# Autodesk Inventor assembly: printer
(part 2 of 2)
- Mate:177: CSN 02 1702 B B 4,3:115 ↔ ISO 4762 M4 x 20:64
- Mate:178: z_rod_stopper_bottom:2 ↔ CSN 02 1702 B B 4,3:119
- Mate:179: CSN 02 1702 B B 4,3:119 ↔ ISO 4762 M4 x 20:63
- Mate:180: z_motor_mount:2 ↔ CSN 02 1702 B B 4,3:128
- Mate:181: CSN 02 1702 B B 4,3:128 ↔ ISO 4762 M4 x 20:60
- Mate:182: z_motor_mount:2 ↔ CSN 02 1702 B B 4,3:118
- Mate:183: CSN 02 1702 B B 4,3:118 ↔ ISO 4762 M4 x 20:58
- Mate:184: brace_right:1 ↔ CSN 02 1702 B B 4,3:126
- Mate:185: CSN 02 1702 B B 4,3:126 ↔ ISO 4762 M4 x 20:62
- Mate:186: z_rod_stopper_bottom:2 ↔ CSN 02 1702 B B 4,3:127
- Mate:187: CSN 02 1702 B B 4,3:127 ↔ ISO 4762 M4 x 20:61
- Mate:188: CSN 02 1702 B B 4,3:119 ↔ DIN EN ISO 7040 M4:51
- Mate:189: ISO 4762 M4 x 20:63 ↔ DIN EN ISO 7040 M4:51
- Mate:190: CSN 02 1702 B B 4,3:115 ↔ DIN EN ISO 7040 M4:54
- Mate:191: ISO 4762 M4 x 20:64 ↔ DIN EN ISO 7040 M4:54
- Mate:192: CSN 02 1702 B B 4,3:125 ↔ DIN EN ISO 7040 M4:52
- Mate:193: ISO 4762 M4 x 20:59 ↔ DIN EN ISO 7040 M4:52
- Mate:194: CSN 02 1702 B B 4,3:128 ↔ DIN EN ISO 7040 M4:53
- Mate:195: ISO 4762 M4 x 20:60 ↔ DIN EN ISO 7040 M4:53
- Mate:196: CSN 02 1702 B B 4,3:118 ↔ DIN EN ISO 7040 M4:55
- Mate:197: ISO 4762 M4 x 20:58 ↔ DIN EN ISO 7040 M4:55
- Mate:198: CSN 02 1702 B B 4,3:126 ↔ DIN EN ISO 7040 M4:50
- Mate:199: ISO 4762 M4 x 20:62 ↔ DIN EN ISO 7040 M4:50
- Mate:200: CSN 02 1702 B B 4,3:127 ↔ DIN EN ISO 7040 M4:49
- Mate:201: ISO 4762 M4 x 20:61 ↔ DIN EN ISO 7040 M4:49
- Mate:202: brace_right:1 ↔ wiring_brace:1
- Mate:203: frame:1 ↔ wiring_brace:1
- Mate:204: brace_right:1 ↔ wiring_brace:1
- Mate:205: brace_left:1 ↔ wiring_brace:2
- Mate:206: frame:1 ↔ wiring_brace:2
- Mate:207: brace_left:1 ↔ wiring_brace:2
- Mate:208: frame:1 ↔ CSN 02 1702 B B 4,3:132
- Mate:209: frame:1 ↔ CSN 02 1702 B B 4,3:132
- Mate:210: wiring_brace:1 ↔ CSN 02 1702 B B 4,3:131
- Mate:211: brace_right:1 ↔ CSN 02 1702 B B 4,3:129
- Mate:212: brace_right:1 ↔ CSN 02 1702 B B 4,3:129
- Mate:213: wiring_brace:1 ↔ CSN 02 1702 B B 4,3:130
- Insert:30: CSN 02 1702 B B 4,3:132 ↔ ISO 4762 M4 x 20:65
- Insert:31: CSN 02 1702 B B 4,3:129 ↔ ISO 4762 M4 x 20:66
- Mate:214: CSN 02 1702 B B 4,3:131 ↔ ISO 4762 M4 x 20:65
- Mate:215: CSN 02 1702 B B 4,3:130 ↔ ISO 4762 M4 x 20:66
- Mate:216: CSN 02 1702 B B 4,3:131 ↔ DIN EN ISO 7040 M4:57
- Mate:217: ISO 4762 M4 x 20:65 ↔ DIN EN ISO 7040 M4:57
- Mate:218: CSN 02 1702 B B 4,3:130 ↔ DIN EN ISO 7040 M4:56
- Mate:219: ISO 4762 M4 x 20:66 ↔ DIN EN ISO 7040 M4:56
- Mate:220: z_motor_mount:2 ↔ CSN 02 1702 B B 3,2:3
- Mate:221: z_motor_mount:2 ↔ CSN 02 1702 B B 3,2:2
- Mate:222: z_motor_mount:2 ↔ CSN 02 1702 B B 3,2:1
- Mate:223: z_motor_mount:2 ↔ CSN 02 1702 B B 3,2:4
- Mate:224: z_motor_mount:2 ↔ CSN 02 1702 B B 3,2:2
- Mate:225: z_motor_mount:2 ↔ CSN 02 1702 B B 3,2:4
- Mate:226: z_motor_mount:2 ↔ CSN 02 1702 B B 3,2:3
- Mate:227: z_motor_mount:2 ↔ CSN 02 1702 B B 3,2:1
- Insert:32: CSN 02 1702 B B 3,2:4 ↔ ISO 4762 M3 x 16:2
- Insert:33: CSN 02 1702 B B 3,2:2 ↔ ISO 4762 M3 x 16:1
- Insert:34: CSN 02 1702 B B 3,2:3 ↔ ISO 4762 M3 x 16:3
- Insert:35: CSN 02 1702 B B 3,2:1 ↔ ISO 4762 M3 x 16:4
- Mate:228: CSN 02 1702 B B 4,3:136 ↔ ISO 4762 M4 x 20:67
- Insert:36: CSN 02 1702 B B 4,3:142 ↔ ISO 4762 M4 x 20:67
- Mate:229: CSN 02 1702 B B 4,3:143 ↔ ISO 4762 M4 x 20:68
- Insert:37: CSN 02 1702 B B 4,3:135 ↔ ISO 4762 M4 x 20:68
- Mate:230: CSN 02 1702 B B 4,3:146 ↔ ISO 4762 M4 x 20:69
- Insert:38: CSN 02 1702 B B 4,3:141 ↔ ISO 4762 M4 x 20:69
- Mate:231: CSN 02 1702 B B 4,3:145 ↔ ISO 4762 M4 x 20:70
- Insert:39: CSN 02 1702 B B 4,3:140 ↔ ISO 4762 M4 x 20:70
- Mate:232: CSN 02 1702 B B 4,3:144 ↔ ISO 4762 M4 x 20:71
- Insert:40: CSN 02 1702 B B 4,3:134 ↔ ISO 4762 M4 x 20:71
- Mate:233: CSN 02 1702 B B 4,3:137 ↔ ISO 4762 M4 x 20:72
- Insert:41: CSN 02 1702 B B 4,3:139 ↔ ISO 4762 M4 x 20:72
- Mate:234: CSN 02 1702 B B 4,3:133 ↔ ISO 4762 M4 x 20:73
- Insert:42: CSN 02 1702 B B 4,3:138 ↔ ISO 4762 M4 x 20:73
- Mate:235: ISO 4762 M4 x 20:70 ↔ DIN EN ISO 7040 M4:58
- Mate:236: CSN 02 1702 B B 4,3:145 ↔ DIN EN ISO 7040 M4:58
- Mate:237: ISO 4762 M4 x 20:71 ↔ DIN EN ISO 7040 M4:59
- Mate:238: CSN 02 1702 B B 4,3:144 ↔ DIN EN ISO 7040 M4:59
- Mate:239: ISO 4762 M4 x 20:72 ↔ DIN EN ISO 7040 M4:60
- Mate:240: CSN 02 1702 B B 4,3:137 ↔ DIN EN ISO 7040 M4:60
- Mate:241: ISO 4762 M4 x 20:68 ↔ DIN EN ISO 7040 M4:61
- Mate:242: CSN 02 1702 B B 4,3:143 ↔ DIN EN ISO 7040 M4:61
- Mate:243: ISO 4762 M4 x 20:69 ↔ DIN EN ISO 7040 M4:62
- Mate:244: CSN 02 1702 B B 4,3:146 ↔ DIN EN ISO 7040 M4:62
- Mate:245: ISO 4762 M4 x 20:73 ↔ DIN EN ISO 7040 M4:63
- Mate:246: CSN 02 1702 B B 4,3:133 ↔ DIN EN ISO 7040 M4:63
- Mate:247: ISO 4762 M4 x 20:67 ↔ DIN EN ISO 7040 M4:64
- Mate:248: CSN 02 1702 B B 4,3:136 ↔ DIN EN ISO 7040 M4:64
- Mate:249: CSN 02 1702 B B 4,3:149 ↔ ISO 4762 M4 x 20:74
- Insert:43: CSN 02 1702 B B 4,3:150 ↔ ISO 4762 M4 x 20:74
- Mate:250: CSN 02 1702 B B 4,3:148 ↔ ISO 4762 M4 x 20:75
- Insert:44: CSN 02 1702 B B 4,3:147 ↔ ISO 4762 M4 x 20:75
- Mate:251: ISO 4762 M4 x 20:75 ↔ DIN EN ISO 7040 M4:65
- Mate:252: CSN 02 1702 B B 4,3:148 ↔ DIN EN ISO 7040 M4:65
- Mate:253: ISO 4762 M4 x 20:74 ↔ DIN EN ISO 7040 M4:66
- Mate:254: CSN 02 1702 B B 4,3:149 ↔ DIN EN ISO 7040 M4:66
- Insert:45: CSN 02 1702 B B 3,2:6 ↔ ISO 4762 M3 x 16:5
- Insert:46: CSN 02 1702 B B 3,2:8 ↔ ISO 4762 M3 x 16:6
- Insert:47: CSN 02 1702 B B 3,2:7 ↔ ISO 4762 M3 x 16:7
- Insert:48: CSN 02 1702 B B 3,2:5 ↔ ISO 4762 M3 x 16:8
- Mate:255: back:1 ↔ PC Fan:1
- Mate:256: back:1 ↔ PC Fan:1
- Mate:257: back:1 ↔ PC Fan:1
- Mate:258 (3 mm): back:1 ↔ User Library-Fan Guard:1
- Mate:259: y_carriage_belt_iddler:2 ↔ y_carriage_belt_iddler_holder:1
- Mate:260: y_carriage_belt_iddler:2 ↔ y_carriage_belt_iddler_holder:1
- Mate:261: y_carriage_belt_iddler:2 ↔ y_carriage_belt_iddler_holder:1
- Mate:262: y_carriage_belt_iddler:1 ↔ y_carriage_belt_iddler_holder:1
- Mate:263: y_carriage_belt_iddler:1 ↔ y_carriage_belt_iddler_holder:1
- Mate:264: y_carriage_belt_iddler:1 ↔ y_carriage_belt_iddler_holder:1
- Mate:265: 608RS:1 ↔ belt_guide:1
- Mate:266: 608RS:1 ↔ belt_guide:1
- Mate:267: belt_guide:1 ↔ belt_guide:2
- Mate:268: belt_guide:1 ↔ belt_guide:2
- Mate:269: 608RS:1 ↔ belt_guide:2
- Mate:270: CSN 02 1702 B B 8,4:5 ↔ CSN 02 1702 B B 8,4:6
- Mate:271: CSN 02 1702 B B 8,4:5 ↔ CSN 02 1702 B B 8,4:6
- Mate:272: CSN 02 1702 B B 8,4:3 ↔ CSN 02 1702 B B 8,4:4
- Mate:273: CSN 02 1702 B B 8,4:3 ↔ CSN 02 1702 B B 8,4:4
- Mate:274: 608RS:1 ↔ CSN 02 1702 B B 8,4:4
- Mate:275: 608RS:1 ↔ CSN 02 1702 B B 8,4:4
- Mate:276: 608RS:1 ↔ CSN 02 1702 B B 8,4:5
- Mate:277: 608RS:1 ↔ CSN 02 1702 B B 8,4:5
- Mate:278: y_carriage_belt_iddler:1 ↔ CSN 02 1702 B B 8,4:6
- Mate:279: y_carriage_belt_iddler:2 ↔ 608RS:1
- Mate:280: y_carriage_belt_iddler:2 ↔ CSN 02 1702 B B 8,4:1
- Mate:281: y_carriage_belt_iddler:2 ↔ CSN 02 1702 B B 8,4:1
- Mate:282: y_carriage_belt_iddler:1 ↔ CSN 02 1702 B B 8,4:2
- Mate:283: y_carriage_belt_iddler:1 ↔ CSN 02 1702 B B 8,4:2
- Insert:49: CSN 02 1702 B B 8,4:2 ↔ ISO 4762 M8 x 40:1
- Mate:284: CSN 02 1702 B B 8,4:1 ↔ DIN EN ISO 7040 M8:1
- Mate:285: ISO 4762 M8 x 40:1 ↔ DIN EN ISO 7040 M8:1
- Mate:286: back:1 ↔ y_carriage_belt_iddler:2
- Mate:287: back:1 ↔ y_carriage_belt_iddler:2
- Mate:288: back:1 ↔ y_carriage_belt_iddler:1
- Mate:289: back:1 ↔ CSN 02 1702 B B 4,3:152
- Mate:290: back:1 ↔ CSN 02 1702 B B 4,3:153
- Mate:291: back:1 ↔ CSN 02 1702 B B 4,3:153
- Mate:292: back:1 ↔ CSN 02 1702 B B 4,3:152
- Insert:50: CSN 02 1702 B B 4,3:152 ↔ ISO 4762 M4 x 30:1
- Insert:51: CSN 02 1702 B B 4,3:153 ↔ ISO 4762 M4 x 30:2
- Mate:293: y_carriage_belt_iddler_holder:1 ↔ CSN 02 1702 B B 4,3:154
- Mate:294: y_carriage_belt_iddler_holder:1 ↔ CSN 02 1702 B B 4,3:151
- Mate:295: CSN 02 1702 B B 4,3:151 ↔ ISO 4762 M4 x 30:2
- Mate:296: CSN 02 1702 B B 4,3:154 ↔ ISO 4762 M4 x 30:1
- Mate:297: CSN 02 1702 B B 4,3:151 ↔ DIN EN ISO 7040 M4:68
- Mate:298: ISO 4762 M4 x 30:2 ↔ DIN EN ISO 7040 M4:68
- Mate:299: CSN 02 1702 B B 4,3:154 ↔ DIN EN ISO 7040 M4:67
- Mate:300: ISO 4762 M4 x 30:1 ↔ DIN EN ISO 7040 M4:67
- Mate:301: y_motor_mount:1 ↔ y_motor_mount_brace:1
- Mate:302: y_motor_mount:1 ↔ y_motor_mount_brace:1
- Mate:303: y_motor_mount:1 ↔ y_motor_mount_brace:1
- Mate:304: front:1 ↔ y_motor_mount:1
- Mate:305: front:1 ↔ y_motor_mount_brace:1
- Mate:306: front:1 ↔ y_motor_mount:1
- Mate:307: front:1 ↔ CSN 02 1702 B B 4,3:159
- Mate:308: front:1 ↔ CSN 02 1702 B B 4,3:160
- Mate:309: front:1 ↔ CSN 02 1702 B B 4,3:160
- Mate:310: front:1 ↔ CSN 02 1702 B B 4,3:159
- Mate:311: y_motor_mount:1 ↔ CSN 02 1702 B B 4,3:157
- Mate:312: y_motor_mount:1 ↔ CSN 02 1702 B B 4,3:157
- Insert:52: CSN 02 1702 B B 4,3:160 ↔ ISO 4762 M4 x 20:78
- Insert:53: CSN 02 1702 B B 4,3:159 ↔ ISO 4762 M4 x 20:77
- Insert:54: CSN 02 1702 B B 4,3:157 ↔ ISO 4762 M4 x 20:76
- Mate:313: y_motor_mount_brace:1 ↔ CSN 02 1702 B B 4,3:158
- Mate:314: CSN 02 1702 B B 4,3:158 ↔ ISO 4762 M4 x 20:78
- Mate:315: y_motor_mount_brace:1 ↔ CSN 02 1702 B B 4,3:155
- Mate:316: CSN 02 1702 B B 4,3:155 ↔ ISO 4762 M4 x 20:76
- Mate:317: y_motor_mount:1 ↔ CSN 02 1702 B B 4,3:156
- Mate:318: CSN 02 1702 B B 4,3:156 ↔ ISO 4762 M4 x 20:77
- Mate:319: CSN 02 1702 B B 4,3:156 ↔ DIN EN ISO 7040 M4:70
- Mate:320: ISO 4762 M4 x 20:77 ↔ DIN EN ISO 7040 M4:70
- Mate:321: CSN 02 1702 B B 4,3:158 ↔ DIN EN ISO 7040 M4:69
- Mate:322: ISO 4762 M4 x 20:78 ↔ DIN EN ISO 7040 M4:69
- Mate:323: CSN 02 1702 B B 4,3:155 ↔ DIN EN ISO 7040 M4:71
- Mate:324: ISO 4762 M4 x 20:76 ↔ DIN EN ISO 7040 M4:71
- Mate:325: motor_spacer:1 ↔ NEMA 17 with T5 Pulley:1
- Mate:326: motor_spacer:1 ↔ NEMA 17 with T5 Pulley:1
- Mate:327: motor_spacer:1 ↔ NEMA 17 with T5 Pulley:1
- Mate:328: y_motor_mount:1 ↔ motor_spacer:1
- Tangent:1: y_motor_mount:1 ↔ motor_spacer:1
- Tangent:2: y_motor_mount:1 ↔ motor_spacer:1
- Mate:329: y_motor_mount:1 ↔ CSN 02 1702 B B 3,2:12
- Mate:330: y_motor_mount:1 ↔ CSN 02 1702 B B 3,2:11
- Mate:331: y_motor_mount:1 ↔ CSN 02 1702 B B 3,2:9
- Mate:332: y_motor_mount:1 ↔ CSN 02 1702 B B 3,2:10
- Insert:55: CSN 02 1702 B B 3,2:12 ↔ ISO 4762 M3 x 16:12
- Insert:56: CSN 02 1702 B B 3,2:11 ↔ ISO 4762 M3 x 16:11
- Insert:57: CSN 02 1702 B B 3,2:9 ↔ ISO 4762 M3 x 16:10
- Insert:58: CSN 02 1702 B B 3,2:10 ↔ ISO 4762 M3 x 16:9
- Mate:333: motor_spacer:1 ↔ ISO 4762 M3 x 16:12
- Mate:334: motor_spacer:1 ↔ ISO 4762 M3 x 16:11
- Mate:335: motor_spacer:1 ↔ ISO 4762 M3 x 16:9
- Mate:336: motor_spacer:1 ↔ ISO 4762 M3 x 16:10
- Mate:337: y_axis_rod:2 ↔ y_carryage:1
- Mate:338: y_axis_rod:1 ↔ y_carryage:1
- Mate:339: z_axis_rod:2 ↔ x_axis:1
- Mate:340: z_axis_rod:1 ↔ x_axis:1
- Mate:341: brace_right:1 ↔ CSN 02 1702 B B 4,3:161
- Mate:342: brace_right:1 ↔ CSN 02 1702 B B 4,3:161
- Insert:59: CSN 02 1702 B B 4,3:161 ↔ ISO 4762 M4 x 20:79
- Mate:343: frame_brace_top:1 ↔ CSN 02 1702 B B 4,3:162
- Mate:344: CSN 02 1702 B B 4,3:162 ↔ ISO 4762 M4 x 20:79
- Mate:345: CSN 02 1702 B B 4,3:162 ↔ DIN EN ISO 7040 M4:72
- Mate:346: ISO 4762 M4 x 20:79 ↔ DIN EN ISO 7040 M4:72
- Mate:347: CSN 02 1702 B B 4,3:164 ↔ ISO 4762 M4 x 20:80
- Insert:60: CSN 02 1702 B B 4,3:163 ↔ ISO 4762 M4 x 20:80
- Mate:348: ISO 4762 M4 x 20:80 ↔ DIN EN ISO 7040 M4:73
- Mate:349: CSN 02 1702 B B 4,3:164 ↔ DIN EN ISO 7040 M4:73
- Mate:350: z_axis_top_cap:2 ↔ CSN 02 1702 B B 4,3:172
- Mate:351: z_axis_top_cap:2 ↔ CSN 02 1702 B B 4,3:174
- Mate:352: z_axis_top_cap:2 ↔ CSN 02 1702 B B 4,3:174
- Mate:353: z_axis_top_cap:2 ↔ CSN 02 1702 B B 4,3:172
- Mate:354: z_axis_top:2 ↔ CSN 02 1702 B B 4,3:173
- Mate:355: z_axis_top:2 ↔ CSN 02 1702 B B 4,3:171
- Mate:356: z_axis_top:2 ↔ CSN 02 1702 B B 4,3:170
- Mate:357: z_axis_top:2 ↔ CSN 02 1702 B B 4,3:170
- Mate:358: z_axis_top:2 ↔ CSN 02 1702 B B 4,3:173
- Mate:359: z_axis_top:2 ↔ CSN 02 1702 B B 4,3:171
- Insert:61: CSN 02 1702 B B 4,3:170 ↔ ISO 4762 M4 x 20:81
- Insert:62: CSN 02 1702 B B 4,3:171 ↔ ISO 4762 M4 x 20:82
- Insert:63: CSN 02 1702 B B 4,3:173 ↔ ISO 4762 M4 x 20:83
- Insert:64: CSN 02 1702 B B 4,3:174 ↔ ISO 4762 M4 x 20:84
- Insert:65: CSN 02 1702 B B 4,3:172 ↔ ISO 4762 M4 x 20:85
- Mate:360: brace_right:1 ↔ CSN 02 1702 B B 4,3:169
- Mate:361: CSN 02 1702 B B 4,3:169 ↔ ISO 4762 M4 x 20:81
- Mate:362: frame:1 ↔ CSN 02 1702 B B 4,3:165
- Mate:363: CSN 02 1702 B B 4,3:165 ↔ ISO 4762 M4 x 20:83
- Mate:364: frame:1 ↔ CSN 02 1702 B B 4,3:166
- Mate:365: CSN 02 1702 B B 4,3:166 ↔ ISO 4762 M4 x 20:82
- Mate:366: z_axis_top:2 ↔ CSN 02 1702 B B 4,3:167
- Mate:367: CSN 02 1702 B B 4,3:167 ↔ ISO 4762 M4 x 20:84
- Mate:368: z_axis_top:2 ↔ CSN 02 1702 B B 4,3:168
- Mate:369: CSN 02 1702 B B 4,3:169 ↔ DIN EN ISO 7040 M4:78
- Mate:370: ISO 4762 M4 x 20:81 ↔ DIN EN ISO 7040 M4:78
- Mate:371: CSN 02 1702 B B 4,3:166 ↔ DIN EN ISO 7040 M4:77
- Mate:372: ISO 4762 M4 x 20:82 ↔ DIN EN ISO 7040 M4:77
- Mate:373: CSN 02 1702 B B 4,3:165 ↔ DIN EN ISO 7040 M4:76
- Mate:374: ISO 4762 M4 x 20:83 ↔ DIN EN ISO 7040 M4:76
- Mate:375: CSN 02 1702 B B 4,3:167 ↔ DIN EN ISO 7040 M4:75
- Mate:376: ISO 4762 M4 x 20:84 ↔ DIN EN ISO 7040 M4:75
- Mate:377: CSN 02 1702 B B 4,3:168 ↔ DIN EN ISO 7040 M4:74
- Mate:378: CSN 02 1702 B B 4,3:168 ↔ ISO 4762 M4 x 20:85
- Mate:379: ISO 4762 M4 x 20:85 ↔ DIN EN ISO 7040 M4:74
- Mate:380: CSN 02 1702 B B 4,3:179 ↔ ISO 4762 M4 x 20:86
- Insert:66: CSN 02 1702 B B 4,3:180 ↔ ISO 4762 M4 x 20:86
- Mate:381: CSN 02 1702 B B 4,3:176 ↔ ISO 4762 M4 x 20:87
- Insert:67: CSN 02 1702 B B 4,3:181 ↔ ISO 4762 M4 x 20:87
- Mate:382: CSN 02 1702 B B 4,3:175 ↔ ISO 4762 M4 x 20:88
- Insert:68: CSN 02 1702 B B 4,3:183 ↔ ISO 4762 M4 x 20:88
- Mate:383: CSN 02 1702 B B 4,3:177 ↔ ISO 4762 M4 x 20:89
- Insert:69: CSN 02 1702 B B 4,3:184 ↔ ISO 4762 M4 x 20:89
- Mate:384: CSN 02 1702 B B 4,3:178 ↔ ISO 4762 M4 x 20:90
- Insert:70: CSN 02 1702 B B 4,3:182 ↔ ISO 4762 M4 x 20:90
- Mate:385: ISO 4762 M4 x 20:90 ↔ DIN EN ISO 7040 M4:79
- Mate:386: CSN 02 1702 B B 4,3:178 ↔ DIN EN ISO 7040 M4:79
- Mate:387: ISO 4762 M4 x 20:89 ↔ DIN EN ISO 7040 M4:80
- Mate:388: CSN 02 1702 B B 4,3:177 ↔ DIN EN ISO 7040 M4:80
- Mate:389: ISO 4762 M4 x 20:88 ↔ DIN EN ISO 7040 M4:81
- Mate:390: CSN 02 1702 B B 4,3:175 ↔ DIN EN ISO 7040 M4:81
- Mate:391: ISO 4762 M4 x 20:87 ↔ DIN EN ISO 7040 M4:82
- Mate:392: CSN 02 1702 B B 4,3:176 ↔ DIN EN ISO 7040 M4:82
- Mate:393: ISO 4762 M4 x 20:86 ↔ DIN EN ISO 7040 M4:83
- Mate:394: CSN 02 1702 B B 4,3:179 ↔ DIN EN ISO 7040 M4:83
- Mate:484: bottom:1 ↔ CSN 02 1702 B B 4,3:213
- Mate:485: bottom:1 ↔ CSN 02 1702 B B 4,3:213
- Insert:85: CSN 02 1702 B B 4,3:213 ↔ ISO 4762 M4 x 20:105
- Mate:486: y_motor_mount:1 ↔ CSN 02 1702 B B 4,3:214
- Mate:487: CSN 02 1702 B B 4,3:214 ↔ ISO 4762 M4 x 20:105
- Mate:488: CSN 02 1702 B B 4,3:214 ↔ DIN EN ISO 7040 M4:98
- Mate:489: ISO 4762 M4 x 20:105 ↔ DIN EN ISO 7040 M4:98
- Mate:500: brace_right:1 ↔ IEC inlet:1
- Mate:501: brace_right:1 ↔ IEC inlet:1
- Mate:502: brace_right:1 ↔ IEC inlet:1
- Mate:503: x_axis:1 ↔ z_axis_cable_mount_b:1
- Mate:504: x_axis:1 ↔ z_axis_cable_mount_b:1
- Mate:505: x_axis:1 ↔ z_axis_cable_mount_b:1
- [Insert]: cable_chain_22:28 ↔ cable_chain_22:29
- [Angle] (-36 deg): cable_chain_22:28 ↔ cable_chain_22:29
- [Insert]: cable_chain_22:29 ↔ cable_chain_22:30
- [Angle] (-36 deg): cable_chain_22:29 ↔ cable_chain_22:30
- [Insert]: cable_chain_22:31 ↔ cable_chain_22:32
- [Angle] (-36 deg): cable_chain_22:31 ↔ cable_chain_22:32
- [Insert]: cable_chain_22:32 ↔ cable_chain_22:33
- [Angle] (-36 deg): cable_chain_22:32 ↔ cable_chain_22:33
- [Insert]: cable_chain_22:34 ↔ cable_chain_22:35
- [Angle] (-36 deg): cable_chain_22:34 ↔ cable_chain_22:35
- [Insert]: cable_chain_22:35 ↔ cable_chain_22:36
- [Angle] (-36 deg): cable_chain_22:35 ↔ cable_chain_22:36
- [Insert]: cable_chain_22:33 ↔ cable_chain_22:34
- [Angle] (-36 deg): cable_chain_22:33 ↔ cable_chain_22:34
- [Insert]: cable_chain_22:30 ↔ cable_chain_22:31
- [Angle] (-36 deg): cable_chain_22:30 ↔ cable_chain_22:31
- [Insert]: cable_chain_22:37 ↔ cable_chain_22:38
- [Angle] (-36 deg): cable_chain_22:37 ↔ cable_chain_22:38
- [Insert]: cable_chain_22:38 ↔ cable_chain_22:39
- [Angle] (-36 deg): cable_chain_22:38 ↔ cable_chain_22:39
- [Insert]: cable_chain_22:40 ↔ cable_chain_22:41
- [Angle] (-36 deg): cable_chain_22:40 ↔ cable_chain_22:41
- [Insert]: cable_chain_22:41 ↔ cable_chain_22:42
- [Angle] (-36 deg): cable_chain_22:41 ↔ cable_chain_22:42
- [Insert]: cable_chain_22:39 ↔ cable_chain_22:40
- [Angle] (-36 deg): cable_chain_22:39 ↔ cable_chain_22:40
- [Insert]: cable_chain_22:43 ↔ cable_chain_22:44
- [Angle] (-36 deg): cable_chain_22:43 ↔ cable_chain_22:44
- [Insert]: cable_chain_22:44 ↔ cable_chain_22:45
- [Angle] (-36 deg): cable_chain_22:44 ↔ cable_chain_22:45
- [Insert]: cable_chain_22:46 ↔ cable_chain_22:47
- [Angle] (-36 deg): cable_chain_22:46 ↔ cable_chain_22:47
- [Insert]: cable_chain_22:47 ↔ cable_chain_22:48
- [Angle] (-36 deg): cable_chain_22:47 ↔ cable_chain_22:48
- [Insert]: cable_chain_22:45 ↔ cable_chain_22:46
- [Angle] (-36 deg): cable_chain_22:45 ↔ cable_chain_22:46
- [Insert]: cable_chain_22:42 ↔ cable_chain_22:43
- [Angle] (-36 deg): cable_chain_22:42 ↔ cable_chain_22:43
- [Insert]: cable_chain_22:36 ↔ cable_chain_22:37
- [Angle] (-36 deg): cable_chain_22:36 ↔ cable_chain_22:37
- Insert:133: z_axis_cable_mount_b:1 ↔ cable_chain_22:48
- Angle:48 (0 deg): z_axis_cable_mount_b:1 ↔ cable_chain_22:48
- Insert:134: cable_chain_22:28 ↔ z_axis_cable_mount_a:1
- Flush:9: cable_chain_22:28 ↔ z_axis_cable_mount_a:1
- Mate:506: brace_left:1 ↔ z_axis_cable_mount_a:1
- Flush:10: brace_left:1 ↔ z_axis_cable_mount_a:1
- Mate:507: y_carryage:1 ↔ y_axis_cable_mount_b:1
- [Insert]: cable_chain_22:77 ↔ cable_chain_22:78
- [Angle] (-36 deg): cable_chain_22:77 ↔ cable_chain_22:78
- [Insert]: cable_chain_22:79 ↔ cable_chain_22:80
- [Angle] (-36 deg): cable_chain_22:79 ↔ cable_chain_22:80
- [Insert]: cable_chain_22:80 ↔ cable_chain_22:81
- [Angle] (-36 deg): cable_chain_22:80 ↔ cable_chain_22:81
- [Insert]: cable_chain_22:82 ↔ cable_chain_22:83
- [Angle] (-36 deg): cable_chain_22:82 ↔ cable_chain_22:83
- [Insert]: cable_chain_22:83 ↔ cable_chain_22:84
- [Angle] (-36 deg): cable_chain_22:83 ↔ cable_chain_22:84
- [Insert]: cable_chain_22:81 ↔ cable_chain_22:82
- [Angle] (-36 deg): cable_chain_22:81 ↔ cable_chain_22:82
- [Insert]: cable_chain_22:78 ↔ cable_chain_22:79
- [Angle] (-36 deg): cable_chain_22:78 ↔ cable_chain_22:79
- [Insert]: cable_chain_22:85 ↔ cable_chain_22:86
- [Angle] (-36 deg): cable_chain_22:85 ↔ cable_chain_22:86
- [Insert]: cable_chain_22:86 ↔ cable_chain_22:87
- [Angle] (-36 deg): cable_chain_22:86 ↔ cable_chain_22:87
- [Insert]: cable_chain_22:88 ↔ cable_chain_22:89
- [Angle] (-36 deg): cable_chain_22:88 ↔ cable_chain_22:89
- [Insert]: cable_chain_22:89 ↔ cable_chain_22:90
- [Angle] (-36 deg): cable_chain_22:89 ↔ cable_chain_22:90
- [Insert]: cable_chain_22:87 ↔ cable_chain_22:88
- [Angle] (-36 deg): cable_chain_22:87 ↔ cable_chain_22:88
- [Insert]: cable_chain_22:91 ↔ cable_chain_22:92
- [Angle] (-36 deg): cable_chain_22:91 ↔ cable_chain_22:92
- [Insert]: cable_chain_22:92 ↔ cable_chain_22:93
- [Angle] (-36 deg): cable_chain_22:92 ↔ cable_chain_22:93
- [Insert]: cable_chain_22:94 ↔ cable_chain_22:95
- [Angle] (-36 deg): cable_chain_22:94 ↔ cable_chain_22:95
- [Insert]: cable_chain_22:95 ↔ cable_chain_22:96
- [Angle] (-36 deg): cable_chain_22:95 ↔ cable_chain_22:96
- [Insert]: cable_chain_22:93 ↔ cable_chain_22:94
- [Angle] (-36 deg): cable_chain_22:93 ↔ cable_chain_22:94
- [Insert]: cable_chain_22:90 ↔ cable_chain_22:91
- [Angle] (-36 deg): cable_chain_22:90 ↔ cable_chain_22:91
- [Insert]: cable_chain_22:84 ↔ cable_chain_22:85
- [Angle] (-36 deg): cable_chain_22:84 ↔ cable_chain_22:85
- Insert:182: y_axis_cable_mount_b:1 ↔ cable_chain_22:96
- Angle:96 (0 deg): y_axis_cable_mount_b:1 ↔ cable_chain_22:96
- Insert:183: cable_chain_22:77 ↔ x_axis_cable_mount_a:1
- Flush:11: cable_chain_22:77 ↔ x_axis_cable_mount_a:1
- Mate:510: bottom:1 ↔ x_axis_cable_mount_a:1
- Mate:511 (90 mm): back:1 ↔ x_axis_cable_mount_a:1
- Flush:12: y_carryage:1 ↔ y_axis_cable_mount_b:1
- Flush:13: y_carryage:1 ↔ y_axis_cable_mount_b:1
- Mate:513: z_threaded_rod:2 ↔ z_axis_coupling_silicone_hose:2
- Mate:514 (-20 mm): NEMA 17:1 ↔ z_axis_coupling_silicone_hose:2
- Mate:515: z_threaded_rod:1 ↔ z_axis_coupling_silicone_hose:1
- Mate:516 (-20 mm): z_threaded_rod:1 ↔ z_axis_coupling_silicone_hose:1
- Mate:517: front:1 ↔ y_axis_cap_front_panel:1
- Mate:518: front:1 ↔ y_axis_cap_front_panel:1
- Mate:519: front:1 ↔ y_axis_cap_front_panel:2
- Mate:520: front:1 ↔ y_axis_cap_front_panel:2
- Angle:97 (0 deg): front:1 ↔ y_axis_cap_front_panel:1
- Angle:98 (0 deg): front:1 ↔ y_axis_cap_front_panel:2
- Mate:521: front:1 ↔ CSN 02 1702 B B 4,3:220
- Mate:522: front:1 ↔ CSN 02 1702 B B 4,3:220
- Mate:523: front:1 ↔ CSN 02 1702 B B 4,3:218
- Mate:524: front:1 ↔ CSN 02 1702 B B 4,3:218
- Mate:525: front:1 ↔ CSN 02 1702 B B 4,3:216
- Mate:526: front:1 ↔ CSN 02 1702 B B 4,3:216
- Mate:527: front:1 ↔ CSN 02 1702 B B 4,3:217
- Mate:528: front:1 ↔ CSN 02 1702 B B 4,3:217
- Insert:184: CSN 02 1702 B B 4,3:220 ↔ ISO 4762 M4 x 20:109
- Insert:185: CSN 02 1702 B B 4,3:218 ↔ ISO 4762 M4 x 20:106
- Insert:186: CSN 02 1702 B B 4,3:216 ↔ ISO 4762 M4 x 20:107
- Insert:187: CSN 02 1702 B B 4,3:217 ↔ ISO 4762 M4 x 20:108
- Mate:529 (5 mm): front:1 ↔ CSN 02 1702 B B 4,3:215
- Mate:530: CSN 02 1702 B B 4,3:215 ↔ ISO 4762 M4 x 20:107
- Mate:531 (5 mm): front:1 ↔ CSN 02 1702 B B 4,3:219
- Mate:532: CSN 02 1702 B B 4,3:219 ↔ ISO 4762 M4 x 20:108
- Mate:533 (5 mm): front:1 ↔ CSN 02 1702 B B 4,3:221
- Mate:534: CSN 02 1702 B B 4,3:221 ↔ ISO 4762 M4 x 20:109
- Mate:535 (5 mm): front:1 ↔ CSN 02 1702 B B 4,3:222
- Mate:536: CSN 02 1702 B B 4,3:222 ↔ ISO 4762 M4 x 20:106
- Mate:537: CSN 02 1702 B B 4,3:215 ↔ DIN EN ISO 7040 M4:100
- Mate:538: ISO 4762 M4 x 20:107 ↔ DIN EN ISO 7040 M4:100
- Mate:539: CSN 02 1702 B B 4,3:219 ↔ DIN EN ISO 7040 M4:99
- Mate:540: ISO 4762 M4 x 20:108 ↔ DIN EN ISO 7040 M4:99
- Mate:541: CSN 02 1702 B B 4,3:221 ↔ DIN EN ISO 7040 M4:101
- Mate:542: ISO 4762 M4 x 20:109 ↔ DIN EN ISO 7040 M4:101
- Mate:543: CSN 02 1702 B B 4,3:222 ↔ DIN EN ISO 7040 M4:102
- Mate:544: ISO 4762 M4 x 20:106 ↔ DIN EN ISO 7040 M4:102
- Mate:545: front:1 ↔ front_panel_2004:1
- Flush:14: front:1 ↔ front_panel_2004:1
- Mate:546: front:1 ↔ front_panel_2004:1
- Mate:547: z_axis_coupling_silicone_hose:2 ↔ coupling_tie:1
- Flush:15 (1.5 mm): z_axis_coupling_silicone_hose:2 ↔ coupling_tie:1
- Flush:16 (1.5 mm): z_axis_coupling_silicone_hose:2 ↔ coupling_tie:3
- Flush:17: coupling_tie:1 ↔ coupling_tie:3
- Mate:548: z_axis_coupling_silicone_hose:2 ↔ coupling_tie:3
- Mate:549: z_axis_coupling_silicone_hose:1 ↔ coupling_tie:4
- Flush:18 (1.5 mm): z_axis_coupling_silicone_hose:1 ↔ coupling_tie:4
- Flush:19 (-1.5 mm): z_axis_coupling_silicone_hose:1 ↔ coupling_tie:2
- Mate:550: z_axis_coupling_silicone_hose:1 ↔ coupling_tie:2
- Flush:20: coupling_tie:2 ↔ coupling_tie:4
- Angle:99 (270 deg): frame:1 ↔ coupling_tie:4
- Angle:100 (90 deg): frame:1 ↔ coupling_tie:1
- Mate:551: coupling_tie:3 ↔ coupling_tie_belt:1
- Mate:552 (1 mm): coupling_tie:3 ↔ coupling_tie_belt:1
- Mate:553 (1 mm): coupling_tie:1 ↔ coupling_tie_belt:2
- Mate:554: coupling_tie:1 ↔ coupling_tie_belt:2
- Mate:555: coupling_tie:2 ↔ coupling_tie_belt:3
- Mate:556 (1 mm): coupling_tie:2 ↔ coupling_tie_belt:3
- Mate:557 (1 mm): coupling_tie:4 ↔ coupling_tie_belt:4
- Mate:558: coupling_tie:4 ↔ coupling_tie_belt:4
- Insert:188: back:1 ↔ Screw F-Z GOST R ISO 7050-93 ST4.2x16-F-Z:6
- Insert:189: back:1 ↔ Screw F-Z GOST R ISO 7050-93 ST4.2x16-F-Z:5
- Insert:190: back:1 ↔ Screw F-Z GOST R ISO 7050-93 ST4.2x16-F-Z:4
- Insert:191: back:1 ↔ Screw F-Z GOST R ISO 7050-93 ST4.2x16-F-Z:3
- Insert:192: IEC inlet:1 ↔ Screw F-Z GOST R ISO 7050-93 ST4.2x16-F-Z:1
- Insert:193: IEC inlet:1 ↔ Screw F-Z GOST R ISO 7050-93 ST4.2x16-F-Z:2
## Named parameters: d552_d406_d403 = -36 deg, d553_d407_d404 = 0 deg, d554_d408_d405 = -36 deg, d555_d409_d389 = -36 deg, d556_d410_d390 = 0 deg, d557_d411_d391 = -36 deg, d558_d412_d392_d389 = -36 deg, d559_d413_d393_d390 = 0 deg, d560_d414_d394_d391 = -36 deg, d561_d415_d395_d382 = 0 mm, d562_d416_d396_d383 = -36 deg, d563_d417_d397_d384 = 0 deg, d564_d418_d398_d385 = -36 deg, d565_d419_d399_d386 = 0 mm, d566_d420_d400_d387 = 0 mm, d567_d421_d401_d388 = 0 mm, d568_d422_d402 = 0 mm, d569_d423_d382 = 0 mm, d570_d424_d383 = -36 deg, d571_d425_d384 = 0 deg, d572_d426_d385 = -36 deg, d573_d427_d386 = 0 mm, d574_d428_d387 = 0 mm, d575_d429_d388 = 0 mm, d576_d430 = 0 mm, d580_d392_d389 = -36 deg, d581_d393_d390 = 0 deg, d582_d394_d391 = -36 deg, d583_d395_d382 = 0 mm, d584_d396_d383 = -36 deg, d585_d397_d384 = 0 deg, d586_d398_d385 = -36 deg, d587_d399_d386 = 0 mm, d588_d400_d387 = 0 mm, d589_d401_d388 = 0 mm, d490_d486 = 0 mm, d491_d487 = -36 deg, d492_d488 = 0 deg, d493_d489 = -36 deg, d494_d431 = -36 deg, d495_d432 = 0 deg, d496_d433 = -36 deg, d497_d434_d431 = -36 deg, d498_d435_d432 = 0 deg, d499_d436_d433 = -36 deg, d500_d437_d403 = -36 deg, d501_d438_d404 = 0 deg, d502_d439_d405 = -36 deg, d503_d440_d406_d403 = -36 deg, d504_d441_d407_d404 = 0 deg, d505_d442_d408_d405 = -36 deg, d506_d443_d409_d389 = -36 deg, d507_d444_d410_d390 = 0 deg, d508_d445_d411_d391 = -36 deg, d509_d446_d412_d392_d389 = -36 deg, d510_d447_d413_d393_d390 = 0 deg, d511_d448_d414_d394_d391 = -36 deg, d512_d449_d415_d395_d382 = 0 mm, d513_d450_d416_d396_d383 = -36 deg, d514_d451_d417_d397_d384 = 0 deg, d515_d452_d418_d398_d385 = -36 deg, d516_d453_d419_d399_d386 = 0 mm, d517_d454_d420_d400_d387 = 0 mm, d518_d455_d421_d401_d388 = 0 mm, d519_d456_d422_d402 = 0 mm, d520_d457_d423_d382 = 0 mm, d521_d458_d424_d383 = -36 deg, d522_d459_d425_d384 = 0 deg, d523_d460_d426_d385 = -36 deg, d524_d461_d427_d386 = 0 mm, d525_d462_d428_d387 = 0 mm, d526_d463_d429_d388 = 0 mm, d527_d464_d430 = 0 mm, d528_d465_d389 = -36 deg, d529_d466_d390 = 0 deg, d530_d467_d391 = -36 deg, d531_d468_d392_d389 = -36 deg, d532_d469_d393_d390 = 0 deg, d533_d470_d394_d391 = -36 deg, d534_d471_d395_d382 = 0 mm, d535_d472_d396_d383 = -36 deg, d536_d473_d397_d384 = 0 deg, d537_d474_d398_d385 = -36 deg, d538_d475_d399_d386 = 0 mm, d539_d476_d400_d387 = 0 mm, d540_d477_d401_d388 = 0 mm, d541_d478_d402 = 0 mm, d542_d479_d382 = 0 mm, d543_d480_d383 = -36 deg, d544_d481_d384 = 0 deg, d545_d482_d385 = -36 deg, d546_d483_d386 = 0 mm, d547_d484_d387 = 0 mm, d548_d485_d388 = 0 mm, d884_d552_d406_d403 = -36 deg, d885_d553_d407_d404 = 0 deg, d886_d554_d408_d405 = -36 deg, d887_d555_d409_d389 = -36 deg, d888_d556_d410_d390 = 0 deg, d889_d557_d411_d391 = -36 deg, d890_d558_d412_d392_d389 = -36 deg, d891_d559_d413_d393_d390 = 0 deg, d892_d560_d414_d394_d391 = -36 deg, d893_d561_d415_d395_d382 = 0 mm, d894_d562_d416_d396_d383 = -36 deg, d895_d563_d417_d397_d384 = 0 deg, d896_d564_d418_d398_d385 = -36 deg, d897_d565_d419_d399_d386 = 0 mm, d898_d566_d420_d400_d387 = 0 mm, d899_d567_d421_d401_d388 = 0 mm, d900_d568_d422_d402 = 0 mm, d901_d569_d423_d382 = 0 mm, d902_d570_d424_d383 = -36 deg, d903_d571_d425_d384 = 0 deg, d904_d572_d426_d385 = -36 deg, d905_d573_d427_d386 = 0 mm, d906_d574_d428_d387 = 0 mm, d907_d575_d429_d388 = 0 mm, d908_d576_d430 = 0 mm, d912_d580_d392_d389 = -36 deg, d913_d581_d393_d390 = 0 deg, d914_d582_d394_d391 = -36 deg, d919_d587_d399_d386 = 0 mm, d920_d588_d400_d387 = 0 mm, d921_d589_d401_d388 = 0 mm, d934_d490_d486 = 0 mm, d935_d491_d487 = -36 deg, d936_d492_d488 = 0 deg, d937_d493_d489 = -36 deg, d938_d494_d431 = -36 deg, d939_d495_d432 = 0 deg, d940_d496_d433 = -36 deg, d941_d497_d434_d431 = -36 deg, d942_d498_d435_d432 = 0 deg, d943_d499_d436_d433 = -36 deg, d944_d500_d437_d403 = -36 deg, d945_d501_d438_d404 = 0 deg, d946_d502_d439_d405 = -36 deg, d947_d503_d440_d406_d403 = -36 deg, d948_d504_d441_d407_d404 = 0 deg, d949_d505_d442_d408_d405 = -36 deg, d950_d506_d443_d409_d389 = -36 deg, d951_d507_d444_d410_d390 = 0 deg, d952_d508_d445_d411_d391 = -36 deg, d953_d509_d446_d412_d392_d389 = -36 deg, d954_d510_d447_d413_d393_d390 = 0 deg, d955_d511_d448_d414_d394_d391 = -36 deg, d956_d512_d449_d415_d395_d382 = 0 mm, d957_d513_d450_d416_d396_d383 = -36 deg, d958_d514_d451_d417_d397_d384 = 0 deg, d959_d515_d452_d418_d398_d385 = -36 deg, d960_d516_d453_d419_d399_d386 = 0 mm, d961_d517_d454_d420_d400_d387 = 0 mm, d962_d518_d455_d421_d401_d388 = 0 mm, d963_d519_d456_d422_d402 = 0 mm, d964_d520_d457_d423_d382 = 0 mm, d965_d521_d458_d424_d383 = -36 deg, d966_d522_d459_d425_d384 = 0 deg, d967_d523_d460_d426_d385 = -36 deg, d968_d524_d461_d427_d386 = 0 mm, d969_d525_d462_d428_d387 = 0 mm, d970_d526_d463_d429_d388 = 0 mm, d971_d527_d464_d430 = 0 mm, d972_d528_d465_d389 = -36 deg, d973_d529_d466_d390 = 0 deg, d974_d530_d467_d391 = -36 deg, d975_d531_d468_d392_d389 = -36 deg, d976_d532_d469_d393_d390 = 0 deg, d977_d533_d470_d394_d391 = -36 deg, d978_d534_d471_d395_d382 = 0 mm, d979_d535_d472_d396_d383 = -36 deg, d980_d536_d473_d397_d384 = 0 deg, d981_d537_d474_d398_d385 = -36 deg, d982_d538_d475_d399_d386 = 0 mm, d983_d539_d476_d400_d387 = 0 mm, d984_d540_d477_d401_d388 = 0 mm, d985_d541_d478_d402 = 0 mm, d986_d542_d479_d382 = 0 mm, d987_d543_d480_d383 = -36 deg, d988_d544_d481_d384 = 0 deg, d989_d545_d482_d385 = -36 deg, d990_d546_d483_d386 = 0 mm, d991_d547_d484_d387 = 0 mm, d992_d548_d485_d388 = 0 mm
